# Autodesk Inventor assembly: nozzle
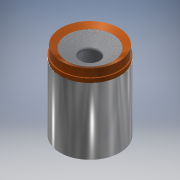
[picture p0: Inventor's stored thumbnail of the model, 180x180]
Saved by Autodesk Inventor 2017 SP1 (Build 210196100, 196)
## iProperties
Created: 2016-10-23
Part Number: nozzle
Document SubType Name: Assembly
Designer: cflannery
Author: cflannery
## Documents named in this file (5)
- D:\Triton_Rocket_Club\NONGIT\Nozzle_designSpace\nozzle.iam
- D:\Triton_Rocket_Club\NONGIT\Nozzle_designSpace\aluminum.ipt
- D:\Triton_Rocket_Club\NONGIT\Nozzle_designSpace\graphite.ipt
- D:\Triton_Rocket_Club\NONGIT\Nozzle_designSpace\pheneolic_bottom.ipt
- D:\Triton_Rocket_Club\NONGIT\Nozzle_designSpace\phenolic_top.ipt
## Components (4 placed, 4 different names)
1. aluminum:1 — Mate:1, Mate:4, Mate:8
2. graphite:1 — Mate:2, Mate:3, Mate:4, Mate:6, Mate:7
3. phenolic_top:1 — Mate:1, Mate:2, Mate:3, Mate:6
4. pheneolic_bottom:1 — Mate:7, Mate:8
## Relationships (7: Mate 7)
- Mate:1: aluminum:1 ↔ phenolic_top:1
- Mate:2: graphite:1 ↔ phenolic_top:1
- Mate:3: graphite:1 ↔ phenolic_top:1
- Mate:4: aluminum:1 ↔ graphite:1
- Mate:6: graphite:1 ↔ phenolic_top:1
- Mate:7: graphite:1 ↔ pheneolic_bottom:1
- Mate:8: aluminum:1 ↔ pheneolic_bottom:1
